# Autodesk Inventor assembly: ASY ДМФ 100 кольцо со шпильками
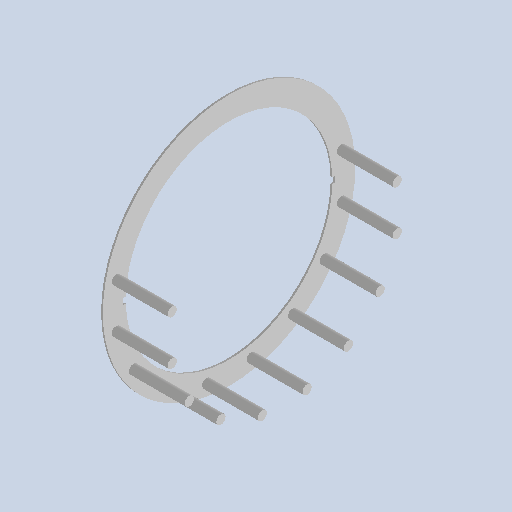
[picture p0: Inventor's stored thumbnail of the model, 512x512]
Saved by Autodesk Inventor 2024.2 (Build 282272000, 272)
## iProperties
Created: 2024-04-23
Part Number: ASY ДМФ 100 кольцо со шпильками
Document SubType Name: Assembly
Designer: admin
Author: admin
## Documents named in this file (4)
- C:\Users\admin\My Drive (bigstupidbeast@gmail.com)\Inventor\Disk Micro filter\DMF-Disk-Micro-Filter\ASY ДМФ 100 кольцо со шпильками.iam
- C:\Users\admin\My Drive (bigstupidbeast@gmail.com)\Inventor\Disk Micro filter\DMF-Disk-Micro-Filter\ДМС 010 кольцо под шпильки.ipt
- C:\Users\admin\My Drive (bigstupidbeast@gmail.com)\Inventor\Disk Micro filter\DMF-Disk-Micro-Filter\ДМС 030 шпилька 1.ipt
- C:\Users\admin\My Drive (bigstupidbeast@gmail.com)\Inventor\Disk Micro filter\DMF-Disk-Micro-Filter\ДМС 000 размеры.ipt
## Components (11 placed, 2 different names)
1. ДМС 010 кольцо под шпильки:1 — Rigid:1, Mate:1
2. ДМС 030 шпилька 1:1 — Rigid:1
3. ДМС 030 шпилька 1:2
4. ДМС 030 шпилька 1:3
5. ДМС 030 шпилька 1:4
6. ДМС 030 шпилька 1:5
7. ДМС 030 шпилька 1:6
8. ДМС 030 шпилька 1:7
9. ДМС 030 шпилька 1:8
10. ДМС 030 шпилька 1:9
11. ДМС 030 шпилька 1:10
## Component patterns: (10 elements, first: ДМС 030 шпилька 1:1)
## Relationships (2: WeldJoint 1, Mate 1)
- Rigid:1 [WeldJoint]: ДМС 010 кольцо под шпильки:1 ↔ ДМС 030 шпилька 1:1
- Mate:1: ДМС 010 кольцо под шпильки:1
